# Autodesk Inventor assembly: Fc Fender Assembly_MIR
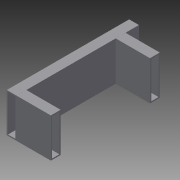
[picture p0: Inventor's stored thumbnail of the model, 180x180]
Saved by Autodesk Inventor 2015 (Build 190159000, 159)
## iProperties
Created: 2015-01-18
Part Number: Fc Fender Assembly_MIR
Document SubType Name: Assembly
Designer: chapale16
Author: chapale16
## Documents named in this file (3)
- \\lhssvr02\Homedirs\Robotics Club\CAD Model 2015\Fc Fender Assembly_MIR.iam
- \\lhssvr02\Homedirs\Robotics Club\CAD Model 2015\4x1 Box Beam 1 ft_MIR.ipt
- \\lhssvr02\Homedirs\Robotics Club\CAD Model 2015\4x1 Box Beam 3.5 in_MIR.ipt
## Components (3 placed, 2 different names)
1. 4x1 Box Beam 1 ft_MIR:1 — Flush:1, Mate:1, Mate:2
2. 4x1 Box Beam 3.5 in_MIR:1 — Flush:1, Mate:1, Mate:3
3. 4x1 Box Beam 3.5 in_MIR:2 — Mate:3, Mate:2
## Relationships (4: Mate 3, Flush 1)
- Flush:1: 4x1 Box Beam 1 ft_MIR:1 ↔ 4x1 Box Beam 3.5 in_MIR:1
- Mate:1: 4x1 Box Beam 1 ft_MIR:1 ↔ 4x1 Box Beam 3.5 in_MIR:1
- Mate:3 (231.8258 mm): 4x1 Box Beam 3.5 in_MIR:1 ↔ 4x1 Box Beam 3.5 in_MIR:2
- Mate:2: 4x1 Box Beam 1 ft_MIR:1 ↔ 4x1 Box Beam 3.5 in_MIR:2
